# Autodesk Inventor assembly: Montagem Lateral
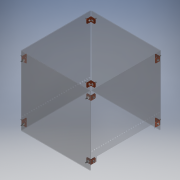
[picture p0: Inventor's stored thumbnail of the model, 180x180]
Saved by Autodesk Inventor 2018 (Build 220112000, 112)
## iProperties
Created: 2018-07-06
Part Number: Montagem Lateral
Material: Genérico
Document SubType Name: Assembly
Designer: Regner
Author: Regner
## Documents named in this file (8)
- C:\Users\Regner\Documents\ROBOTA\2018\Tortura Ratos\Montagem Lateral.iam
- C:\Users\Regner\Documents\ROBOTA\2018\Tortura Ratos\Lateral Acrilico.ipt
- C:\Users\Regner\Documents\Inventor\Content Center Files\R2018\pt-BR\AS 1112 (4)\AS 1112 - M4(2).ipt
- C:\Users\Regner\Documents\ROBOTA\2018\Tortura Ratos\Cantoneira.ipt
- C:\Users\Regner\Documents\Inventor\Content Center Files\R2018\pt-BR\GB_T 822-2000 H\Screw GB_T 822 M4 x 16.ipt
- C:\Users\Regner\Documents\ROBOTA\2018\Tortura Ratos\Frente Acrilico.ipt
- C:\Users\Regner\Documents\Inventor\Content Center Files\R2018\pt-BR\GB_T 822-2000 H\Screw GB_T 822 M4 x 8.ipt
- C:\Users\Regner\Documents\ROBOTA\2018\Tortura Ratos\Lateral Acrilico Furada.ipt
## Components (59 placed, 7 different names)
1. Lateral Acrilico Furada:1 — Coincidência:175, Coincidência:176, Coincidência:177, Coincidência:178, Coincidência:179, Coincidência:181, Coincidência:187, Coincidência:194, Coincidência:195
2. Lateral Acrilico Furada:2 — Coincidência:188, Coincidência:189, Coincidência:190, Coincidência:191, Coincidência:192, Coincidência:193, Coincidência:196
3. Screw GB/T 822-2000 Type H M4 x 16:1 — Coincidência:26, Coincidência:36, Coincidência:54, Coincidência:170
4. Screw GB/T 822-2000 Type H M4 x 16:4 — Coincidência:24, Coincidência:43, Coincidência:46, Coincidência:178
5. Screw GB/T 822-2000 Type H M4 x 16:3 — Coincidência:25, Coincidência:41, Coincidência:53, Coincidência:189
6. Screw GB/T 822-2000 Type H M4 x 16:2 — Coincidência:27, Coincidência:42, Coincidência:57
7. AS 1112 (4) - Métrica M4:1 — Coincidência:20, Coincidência:198
8. AS 1112 (4) - Métrica M4:2 — Coincidência:41, Coincidência:187, Coincidência:188
9. AS 1112 (4) - Métrica M4:3 — Coincidência:36, Coincidência:184
10. AS 1112 (4) - Métrica M4:4 — Coincidência:43, Coincidência:195
11. AS 1112 (4) - Métrica M4:5 — Coincidência:14, Coincidência:191
12. AS 1112 (4) - Métrica M4:6 — Coincidência:17, Coincidência:196
13. AS 1112 (4) - Métrica M4:7 — Coincidência:42, Coincidência:181
14. AS 1112 (4) - Métrica M4:8 — Coincidência:15, Coincidência:192
15. Cantoneira:1 — Coincidência:20, Coincidência:26, Coincidência:54, Coincidência:66, Coincidência:72, Coincidência:169
16. Cantoneira:2 — Coincidência:17, Coincidência:24, Coincidência:46, Coincidência:82, Coincidência:83, Coincidência:90, Coincidência:179
17. Cantoneira:3 — Coincidência:14, Coincidência:27, Coincidência:57, Coincidência:61, Coincidência:63, Coincidência:64, Coincidência:168, Coincidência:175
18. Cantoneira:4 — Coincidência:15, Coincidência:25, Coincidência:53, Coincidência:84, Coincidência:85, Coincidência:165, Coincidência:176
19. Lateral Acrilico:3 — Coincidência:61, Alinhamento:8, Alinhamento:9, Coincidência:180, Coincidência:182, Coincidência:183, Coincidência:184, Coincidência:185
20. Lateral Acrilico:4 — Coincidência:75, Coincidência:86, Coincidência:87, Coincidência:166, Coincidência:168, Coincidência:169, Coincidência:170, Coincidência:171, Coincidência:174, Coincidência:186, Coincidência:197
21. Screw GB/T 822-2000 Type H M4 x 16:5 — Coincidência:63, Coincidência:64, Coincidência:65, Coincidência:69, Coincidência:75
22. Screw GB/T 822-2000 Type H M4 x 16:6 — Coincidência:66, Coincidência:67, Coincidência:68, Coincidência:72, Coincidência:177, Coincidência:190
23. AS 1112 (4) - Métrica M4:9 — Coincidência:69, Coincidência:186
24. AS 1112 (4) - Métrica M4:10 — Coincidência:68, Coincidência:193
25. AS 1112 (4) - Métrica M4:11 — Coincidência:67, Coincidência:194
26. AS 1112 (4) - Métrica M4:12 — Coincidência:65, Coincidência:185
27. AS 1112 (4) - Métrica M4:13 — Coincidência:88, Coincidência:113, Coincidência:183
28. AS 1112 (4) - Métrica M4:14 — Coincidência:115, Coincidência:182
29. AS 1112 (4) - Métrica M4:15 — Coincidência:88, Coincidência:197
30. AS 1112 (4) - Métrica M4:16 — Coincidência:86, Coincidência:87, Coincidência:180
31. Screw GB/T 822-2000 Type H M4 x 16:7 — Coincidência:82, Coincidência:83, Coincidência:91, Coincidência:95, Coincidência:102, Coincidência:106
32. Screw GB/T 822-2000 Type H M4 x 16:8 — Coincidência:84, Coincidência:85, Coincidência:92, Coincidência:93, Coincidência:103, Coincidência:104
33. Lateral Acrilico:5 — Coincidência:90, Coincidência:91, Coincidência:92, Coincidência:94, Coincidência:96, Coincidência:97, Coincidência:98, Coincidência:99, Coincidência:100, Coincidência:116, Coincidência:118, Alinhamento:6, Alinhamento:7, Coincidência:165, Coincidência:198
34. Lateral Acrilico:6 — Coincidência:101, Coincidência:102, Coincidência:103, Coincidência:105, Coincidência:107, Coincidência:109, Coincidência:111
35. AS 1112 (4) - Métrica M4:17 — Coincidência:99, Coincidência:100, Coincidência:110, Coincidência:117
36. AS 1112 (4) - Métrica M4:18 — Coincidência:95, Coincidência:96, Coincidência:101
37. AS 1112 (4) - Métrica M4:19 — Coincidência:93, Coincidência:94
38. AS 1112 (4) - Métrica M4:20 — Coincidência:97, Coincidência:98, Coincidência:108, Coincidência:119
39. AS 1112 (4) - Métrica M4:21 — Coincidência:108, Coincidência:109
40. AS 1112 (4) - Métrica M4:22 — Coincidência:106, Coincidência:107
41. AS 1112 (4) - Métrica M4:23 — Coincidência:110, Coincidência:111
42. AS 1112 (4) - Métrica M4:24 — Coincidência:104, Coincidência:105
43. Cantoneira:5 — Coincidência:116, Coincidência:117, Alinhamento:7, Coincidência:123, Coincidência:130, Coincidência:131, Coincidência:138
44. Cantoneira:6 — Coincidência:115, Alinhamento:8, Coincidência:125, Coincidência:128, Coincidência:134, Coincidência:135, Coincidência:166
45. Cantoneira:7 — Coincidência:113, Alinhamento:9, Coincidência:120, Coincidência:122, Coincidência:124, Coincidência:129, Coincidência:136, Coincidência:137, Coincidência:174
46. Cantoneira:8 — Coincidência:118, Coincidência:119, Alinhamento:6, Coincidência:121, Coincidência:126, Coincidência:127, Coincidência:132, Coincidência:133, Coincidência:147
47. Frente Acrilico:1 — Coincidência:120, Coincidência:121, Coincidência:122, Coincidência:140, Coincidência:142, Coincidência:144, Coincidência:146, Coincidência:147, Coincidência:148, Coincidência:149, Alinhamento:10, Alinhamento:11, Alinhamento:12
48. Screw GB/T 822-2000 Type H M4 x 8:1 — Coincidência:125, Coincidência:128, Coincidência:143, Coincidência:149
49. Screw GB/T 822-2000 Type H M4 x 8:2 — Coincidência:126, Coincidência:127, Coincidência:145
50. Screw GB/T 822-2000 Type H M4 x 8:3 — Coincidência:124, Coincidência:129, Coincidência:139
51. Screw GB/T 822-2000 Type H M4 x 8:4 — Coincidência:123, Coincidência:130, Coincidência:141, Coincidência:148
52. Screw GB/T 822-2000 Type H M4 x 16:9 — Coincidência:132, Coincidência:133
53. Screw GB/T 822-2000 Type H M4 x 16:10 — Coincidência:131, Coincidência:138
54. Screw GB/T 822-2000 Type H M4 x 16:11 — Coincidência:134, Coincidência:135
55. Screw GB/T 822-2000 Type H M4 x 16:12 — Coincidência:136, Coincidência:137, Coincidência:171
56. AS 1112 (4) - Métrica M4:25 — Coincidência:139, Coincidência:140
57. AS 1112 (4) - Métrica M4:26 — Coincidência:143, Coincidência:144
58. AS 1112 (4) - Métrica M4:27 — Coincidência:145, Coincidência:146
59. AS 1112 (4) - Métrica M4:28 — Coincidência:141, Coincidência:142
## Relationships (129: Mate 122, Flush 7)
- Coincidência:14 [Mate]: AS 1112 (4) - Métrica M4:5 ↔ Cantoneira:3
- Coincidência:15 [Mate]: AS 1112 (4) - Métrica M4:8 ↔ Cantoneira:4
- Coincidência:17 [Mate]: AS 1112 (4) - Métrica M4:6 ↔ Cantoneira:2
- Coincidência:20 [Mate]: AS 1112 (4) - Métrica M4:1 ↔ Cantoneira:1
- Coincidência:24 [Mate]: Screw GB/T 822-2000 Type H M4 x 16:4 ↔ Cantoneira:2
- Coincidência:25 [Mate]: Screw GB/T 822-2000 Type H M4 x 16:3 ↔ Cantoneira:4
- Coincidência:26 [Mate]: Screw GB/T 822-2000 Type H M4 x 16:1 ↔ Cantoneira:1
- Coincidência:27 [Mate]: Screw GB/T 822-2000 Type H M4 x 16:2 ↔ Cantoneira:3
- Coincidência:36 [Mate]: Screw GB/T 822-2000 Type H M4 x 16:1 ↔ AS 1112 (4) - Métrica M4:3
- Coincidência:41 [Mate]: Screw GB/T 822-2000 Type H M4 x 16:3 ↔ AS 1112 (4) - Métrica M4:2
- Coincidência:42 [Mate]: Screw GB/T 822-2000 Type H M4 x 16:2 ↔ AS 1112 (4) - Métrica M4:7
- Coincidência:43 [Mate]: Screw GB/T 822-2000 Type H M4 x 16:4 ↔ AS 1112 (4) - Métrica M4:4
- Coincidência:46 [Mate]: Screw GB/T 822-2000 Type H M4 x 16:4 ↔ Cantoneira:2
- Coincidência:53 [Mate]: Screw GB/T 822-2000 Type H M4 x 16:3 ↔ Cantoneira:4
- Coincidência:54 [Mate]: Screw GB/T 822-2000 Type H M4 x 16:1 ↔ Cantoneira:1
- Coincidência:57 [Mate]: Screw GB/T 822-2000 Type H M4 x 16:2 ↔ Cantoneira:3
- Coincidência:61 [Mate]: Cantoneira:3 ↔ Lateral Acrilico:3
- Coincidência:63 [Mate]: Cantoneira:3 ↔ Screw GB/T 822-2000 Type H M4 x 16:5
- Coincidência:64 [Mate]: Cantoneira:3 ↔ Screw GB/T 822-2000 Type H M4 x 16:5
- Coincidência:65 [Mate]: Screw GB/T 822-2000 Type H M4 x 16:5 ↔ AS 1112 (4) - Métrica M4:12
- Coincidência:66 [Mate]: Cantoneira:1 ↔ Screw GB/T 822-2000 Type H M4 x 16:6
- Coincidência:67 [Mate]: Screw GB/T 822-2000 Type H M4 x 16:6 ↔ AS 1112 (4) - Métrica M4:11
- Coincidência:68 [Mate]: Screw GB/T 822-2000 Type H M4 x 16:6 ↔ AS 1112 (4) - Métrica M4:10
- Coincidência:69 [Mate]: Screw GB/T 822-2000 Type H M4 x 16:5 ↔ AS 1112 (4) - Métrica M4:9
- Coincidência:72 [Mate]: Cantoneira:1 ↔ Screw GB/T 822-2000 Type H M4 x 16:6
- Coincidência:75 [Mate]: Lateral Acrilico:4 ↔ Screw GB/T 822-2000 Type H M4 x 16:5
- Coincidência:82 [Mate]: Cantoneira:2 ↔ Screw GB/T 822-2000 Type H M4 x 16:7
- Coincidência:83 [Mate]: Cantoneira:2 ↔ Screw GB/T 822-2000 Type H M4 x 16:7
- Coincidência:84 [Mate]: Cantoneira:4 ↔ Screw GB/T 822-2000 Type H M4 x 16:8
- Coincidência:85 [Mate]: Cantoneira:4 ↔ Screw GB/T 822-2000 Type H M4 x 16:8
- Coincidência:86 [Mate]: Lateral Acrilico:4 ↔ AS 1112 (4) - Métrica M4:16
- Coincidência:87 [Mate]: Lateral Acrilico:4 ↔ AS 1112 (4) - Métrica M4:16
- Coincidência:88 [Mate]: AS 1112 (4) - Métrica M4:13 ↔ AS 1112 (4) - Métrica M4:15
- Coincidência:90 [Mate]: Cantoneira:2 ↔ Lateral Acrilico:5
- Coincidência:91 [Mate]: Screw GB/T 822-2000 Type H M4 x 16:7 ↔ Lateral Acrilico:5
- Coincidência:92 [Mate]: Screw GB/T 822-2000 Type H M4 x 16:8 ↔ Lateral Acrilico:5
- Coincidência:93 [Mate]: Screw GB/T 822-2000 Type H M4 x 16:8 ↔ AS 1112 (4) - Métrica M4:19
- Coincidência:94 [Mate]: Lateral Acrilico:5 ↔ AS 1112 (4) - Métrica M4:19
- Coincidência:95 [Mate]: Screw GB/T 822-2000 Type H M4 x 16:7 ↔ AS 1112 (4) - Métrica M4:18
- Coincidência:96 [Mate]: Lateral Acrilico:5 ↔ AS 1112 (4) - Métrica M4:18
- Coincidência:97 [Mate]: Lateral Acrilico:5 ↔ AS 1112 (4) - Métrica M4:20
- Coincidência:98 [Mate]: Lateral Acrilico:5 ↔ AS 1112 (4) - Métrica M4:20
- Coincidência:99 [Mate]: Lateral Acrilico:5 ↔ AS 1112 (4) - Métrica M4:17
- Coincidência:100 [Mate]: Lateral Acrilico:5 ↔ AS 1112 (4) - Métrica M4:17
- Coincidência:101 [Mate]: Lateral Acrilico:6 ↔ AS 1112 (4) - Métrica M4:18
- Coincidência:102 [Mate]: Screw GB/T 822-2000 Type H M4 x 16:7 ↔ Lateral Acrilico:6
- Coincidência:103 [Mate]: Screw GB/T 822-2000 Type H M4 x 16:8 ↔ Lateral Acrilico:6
- Coincidência:104 [Mate]: Screw GB/T 822-2000 Type H M4 x 16:8 ↔ AS 1112 (4) - Métrica M4:24
- Coincidência:105 [Mate]: Lateral Acrilico:6 ↔ AS 1112 (4) - Métrica M4:24
- Coincidência:106 [Mate]: Screw GB/T 822-2000 Type H M4 x 16:7 ↔ AS 1112 (4) - Métrica M4:22
- Coincidência:107 [Mate]: Lateral Acrilico:6 ↔ AS 1112 (4) - Métrica M4:22
- Coincidência:108 [Mate]: AS 1112 (4) - Métrica M4:20 ↔ AS 1112 (4) - Métrica M4:21
- Coincidência:109 [Mate]: Lateral Acrilico:6 ↔ AS 1112 (4) - Métrica M4:21
- Coincidência:110 [Mate]: AS 1112 (4) - Métrica M4:17 ↔ AS 1112 (4) - Métrica M4:23
- Coincidência:111 [Mate]: Lateral Acrilico:6 ↔ AS 1112 (4) - Métrica M4:23
- Coincidência:113 [Mate]: AS 1112 (4) - Métrica M4:13 ↔ Cantoneira:7
- Coincidência:115 [Mate]: AS 1112 (4) - Métrica M4:14 ↔ Cantoneira:6
- Coincidência:116 [Mate]: Lateral Acrilico:5 ↔ Cantoneira:5
- Coincidência:117 [Mate]: AS 1112 (4) - Métrica M4:17 ↔ Cantoneira:5
- Coincidência:118 [Mate]: Lateral Acrilico:5 ↔ Cantoneira:8
- Coincidência:119 [Mate]: AS 1112 (4) - Métrica M4:20 ↔ Cantoneira:8
- Alinhamento:6 [Flush]: Lateral Acrilico:5 ↔ Cantoneira:8
- Alinhamento:7 [Flush]: Lateral Acrilico:5 ↔ Cantoneira:5
- Alinhamento:8 [Flush]: Lateral Acrilico:3 ↔ Cantoneira:6
- Alinhamento:9 [Flush]: Lateral Acrilico:3 ↔ Cantoneira:7
- Coincidência:120 [Mate]: Cantoneira:7 ↔ Frente Acrilico:1
- Coincidência:121 [Mate]: Cantoneira:8 ↔ Frente Acrilico:1
- Coincidência:122 [Mate]: Cantoneira:7 ↔ Frente Acrilico:1
- Coincidência:123 [Mate]: Cantoneira:5 ↔ Screw GB/T 822-2000 Type H M4 x 8:4
- Coincidência:124 [Mate]: Cantoneira:7 ↔ Screw GB/T 822-2000 Type H M4 x 8:3
- Coincidência:125 [Mate]: Cantoneira:6 ↔ Screw GB/T 822-2000 Type H M4 x 8:1
- Coincidência:126 [Mate]: Cantoneira:8 ↔ Screw GB/T 822-2000 Type H M4 x 8:2
- Coincidência:127 [Mate]: Cantoneira:8 ↔ Screw GB/T 822-2000 Type H M4 x 8:2
- Coincidência:128 [Mate]: Cantoneira:6 ↔ Screw GB/T 822-2000 Type H M4 x 8:1
- Coincidência:129 [Mate]: Cantoneira:7 ↔ Screw GB/T 822-2000 Type H M4 x 8:3
- Coincidência:130 [Mate]: Cantoneira:5 ↔ Screw GB/T 822-2000 Type H M4 x 8:4
- Coincidência:131 [Mate]: Cantoneira:5 ↔ Screw GB/T 822-2000 Type H M4 x 16:10
- Coincidência:132 [Mate]: Cantoneira:8 ↔ Screw GB/T 822-2000 Type H M4 x 16:9
- Coincidência:133 [Mate]: Cantoneira:8 ↔ Screw GB/T 822-2000 Type H M4 x 16:9
- Coincidência:134 [Mate]: Cantoneira:6 ↔ Screw GB/T 822-2000 Type H M4 x 16:11
- Coincidência:135 [Mate]: Cantoneira:6 ↔ Screw GB/T 822-2000 Type H M4 x 16:11
- Coincidência:136 [Mate]: Cantoneira:7 ↔ Screw GB/T 822-2000 Type H M4 x 16:12
- Coincidência:137 [Mate]: Cantoneira:7 ↔ Screw GB/T 822-2000 Type H M4 x 16:12
- Coincidência:138 [Mate]: Cantoneira:5 ↔ Screw GB/T 822-2000 Type H M4 x 16:10
- Coincidência:139 [Mate]: Screw GB/T 822-2000 Type H M4 x 8:3 ↔ AS 1112 (4) - Métrica M4:25
- Coincidência:140 [Mate]: Frente Acrilico:1 ↔ AS 1112 (4) - Métrica M4:25
- Coincidência:141 [Mate]: Screw GB/T 822-2000 Type H M4 x 8:4 ↔ AS 1112 (4) - Métrica M4:28
- Coincidência:142 [Mate]: Frente Acrilico:1 ↔ AS 1112 (4) - Métrica M4:28
- Coincidência:143 [Mate]: Screw GB/T 822-2000 Type H M4 x 8:1 ↔ AS 1112 (4) - Métrica M4:26
- Coincidência:144 [Mate]: Frente Acrilico:1 ↔ AS 1112 (4) - Métrica M4:26
- Coincidência:145 [Mate]: Screw GB/T 822-2000 Type H M4 x 8:2 ↔ AS 1112 (4) - Métrica M4:27
- Coincidência:146 [Mate]: Frente Acrilico:1 ↔ AS 1112 (4) - Métrica M4:27
- Coincidência:147 [Mate]: Cantoneira:8 ↔ Frente Acrilico:1
- Coincidência:148 [Mate]: Frente Acrilico:1 ↔ Screw GB/T 822-2000 Type H M4 x 8:4
- Coincidência:149 [Mate]: Frente Acrilico:1 ↔ Screw GB/T 822-2000 Type H M4 x 8:1
- Coincidência:165 [Mate]: Cantoneira:4 ↔ Lateral Acrilico:5
- Alinhamento:10 [Flush]: Frente Acrilico:1
- Alinhamento:11 [Flush]: Frente Acrilico:1
- Alinhamento:12 [Flush]: Frente Acrilico:1
- Coincidência:166 [Mate]: Lateral Acrilico:4 ↔ Cantoneira:6
- Coincidência:168 [Mate]: Cantoneira:3 ↔ Lateral Acrilico:4
- Coincidência:169 [Mate]: Cantoneira:1 ↔ Lateral Acrilico:4
- Coincidência:170 [Mate]: Screw GB/T 822-2000 Type H M4 x 16:1 ↔ Lateral Acrilico:4
- Coincidência:171 [Mate]: Lateral Acrilico:4 ↔ Screw GB/T 822-2000 Type H M4 x 16:12
- Coincidência:174 [Mate]: Lateral Acrilico:4 ↔ Cantoneira:7
- Coincidência:175 [Mate]: Lateral Acrilico Furada:1 ↔ Cantoneira:3
- Coincidência:176 [Mate]: Lateral Acrilico Furada:1 ↔ Cantoneira:4
- Coincidência:177 [Mate]: Lateral Acrilico Furada:1 ↔ Screw GB/T 822-2000 Type H M4 x 16:6
- Coincidência:178 [Mate]: Lateral Acrilico Furada:1 ↔ Screw GB/T 822-2000 Type H M4 x 16:4
- Coincidência:179 [Mate]: Lateral Acrilico Furada:1 ↔ Cantoneira:2
- Coincidência:180 [Mate]: Lateral Acrilico:3 ↔ AS 1112 (4) - Métrica M4:16
- Coincidência:181 [Mate]: Lateral Acrilico Furada:1 ↔ AS 1112 (4) - Métrica M4:7
- Coincidência:182 [Mate]: Lateral Acrilico:3 ↔ AS 1112 (4) - Métrica M4:14
- Coincidência:183 [Mate]: Lateral Acrilico:3 ↔ AS 1112 (4) - Métrica M4:13
- Coincidência:184 [Mate]: AS 1112 (4) - Métrica M4:3 ↔ Lateral Acrilico:3
- Coincidência:185 [Mate]: Lateral Acrilico:3 ↔ AS 1112 (4) - Métrica M4:12
- Coincidência:186 [Mate]: Lateral Acrilico:4 ↔ AS 1112 (4) - Métrica M4:9
- Coincidência:187 [Mate]: Lateral Acrilico Furada:1 ↔ AS 1112 (4) - Métrica M4:2
- Coincidência:188 [Mate]: Lateral Acrilico Furada:2 ↔ AS 1112 (4) - Métrica M4:2
- Coincidência:189 [Mate]: Lateral Acrilico Furada:2 ↔ Screw GB/T 822-2000 Type H M4 x 16:3
- Coincidência:190 [Mate]: Lateral Acrilico Furada:2 ↔ Screw GB/T 822-2000 Type H M4 x 16:6
- Coincidência:191 [Mate]: Lateral Acrilico Furada:2 ↔ AS 1112 (4) - Métrica M4:5
- Coincidência:192 [Mate]: Lateral Acrilico Furada:2 ↔ AS 1112 (4) - Métrica M4:8
- Coincidência:193 [Mate]: Lateral Acrilico Furada:2 ↔ AS 1112 (4) - Métrica M4:10
- Coincidência:194 [Mate]: Lateral Acrilico Furada:1 ↔ AS 1112 (4) - Métrica M4:11
- Coincidência:195 [Mate]: Lateral Acrilico Furada:1 ↔ AS 1112 (4) - Métrica M4:4
- Coincidência:196 [Mate]: Lateral Acrilico Furada:2 ↔ AS 1112 (4) - Métrica M4:6
- Coincidência:197 [Mate]: Lateral Acrilico:4 ↔ AS 1112 (4) - Métrica M4:15
- Coincidência:198 [Mate]: AS 1112 (4) - Métrica M4:1 ↔ Lateral Acrilico:5
